# Autodesk Inventor assembly: FMS90mm12BladeMotor
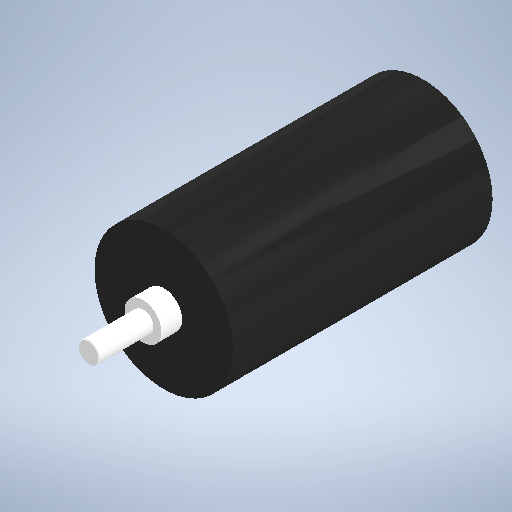
[picture p0: Inventor's stored thumbnail of the model, 512x512]
Saved by Autodesk Inventor 2026.2 (Build 302298010, 298A)
## iProperties
Created: 2026-03-10
Part Number: FMS90mm12BladeMotor
Document SubType Name: Assembly
Designer: tngzj
Author: tngzj
## Documents named in this file (4)
- C:\Transformer-rl-retro-propulsion\CAD\v1\References\FMS90mm12Blade8SAssly v7\FMS90mm12Blade8SAssly v7\FMS90mm12BladeMotor v4.iam
- C:\Transformer-rl-retro-propulsion\CAD\v1\References\FMS90mm12Blade8SAssly v7\FMS90mm12Blade8SAssly v7\Component1_1.ipt
- C:\Transformer-rl-retro-propulsion\CAD\v1\References\FMS90mm12Blade8SAssly v7\FMS90mm12Blade8SAssly v7\Component2_1.ipt
- C:\Transformer-rl-retro-propulsion\CAD\v1\References\FMS90mm12Blade8SAssly v7\FMS90mm12Blade8SAssly v7\Part10.ipt
## Components (3 placed, 3 different names)
1. Component1:1 — Mate:2, Mate:3, Mate:4
2. Component2:1 — Mate:1, Mate:2
3. Part10 — Mate:1, Mate:3, Mate:4
## Relationships (4: Mate 4)
- Mate:1: Component2:1 ↔ Part10
- Mate:2: Component1:1 ↔ Component2:1
- Mate:3: Component1:1 ↔ Part10
- Mate:4: Component1:1 ↔ Part10
